# Autodesk Inventor assembly: ヘッケン＋揺動節2_MIR
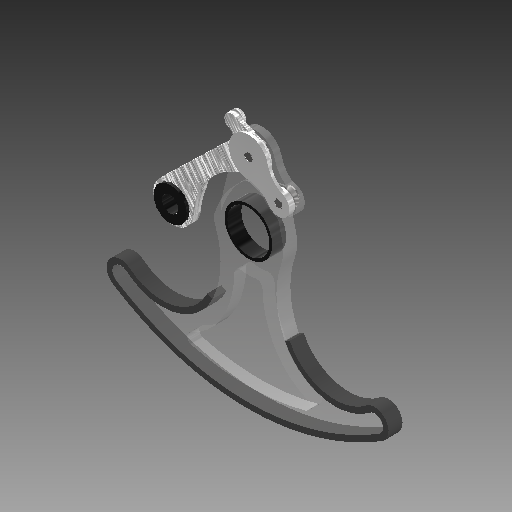
[picture p0: Inventor's stored thumbnail of the model, 512x512]
Saved by Autodesk Inventor 2020 (Build 240168000, 168)
## iProperties
Created: 2019-09-03
Part Number: ヘッケン＋揺動節2_MIR
Document SubType Name: Assembly
Designer: 雪村
Mass: 16.6288 g
Surface Area: 132.4 cm^2
Volume: 11.4961 cm^3
Density: 1.44647 g/cm^3
Author: 雪村
## Documents named in this file (9)
- C:\Users\white\Documents\SRDC\SRDC\Inventor_2017\2018年機体\2020年4年機体\ヘッケン＋揺動節2_MIR.iam
- C:\Users\white\Documents\SRDC\SRDC\Inventor_2017\2018年機体\パーツ\オイレス151705.ipt
- C:\Users\white\Documents\SRDC\SRDC\Inventor_2017\2018年機体\2020年4年機体\ヘッケン2_MIR.ipt
- C:\Users\white\Documents\SRDC\SRDC\Inventor_2017\2018年機体\2020年4年機体\脚揺動節1_MIR1.ipt
- C:\Users\white\Documents\SRDC\SRDC\Inventor_2017\2018年機体\2020年4年機体\脚ゴム2.ipt
- C:\Users\white\Documents\SRDC\SRDC\Inventor_2017\2018年機体\2020年4年機体\脚揺動節抑え1.ipt
- C:\Users\white\Documents\SRDC\SRDC\Inventor_2017\2018年機体\パーツ\オイレス060801.5.ipt
- C:\Users\white\Documents\SRDC\SRDC\Inventor_2017\2018年機体\パーツ\ネジ皿m3,05.ipt
- C:\Users\white\Documents\SRDC\SRDC\Inventor_2017\2018年機体\パーツ\オイレスフランジ付き06080512,1t.ipt
## Components (9 placed, 8 different names)
1. オイレス151705:1 — 挿入:4
2. ヘッケン2_MIR:1 — 挿入:1, 挿入:2, 挿入:4, 挿入:5, 挿入:6, 挿入:7, 挿入:8, 挿入:9
3. 脚揺動節1_MIR1:1 — 挿入:3, 挿入:10
4. 脚ゴム2:1 — 挿入:1, 挿入:2
5. 脚揺動節抑え1:1 — 挿入:6, 挿入:7
6. オイレス060801.5:1 — 挿入:3, 挿入:5
7. ネジ皿m3,05:1 — 挿入:8
8. ネジ皿m3,05:2 — 挿入:9
9. オイレスフランジ付き06080512,1t:1 — 挿入:10
## Relationships (10: Insert 10)
- 挿入:1 [Insert]: ヘッケン2_MIR:1 ↔ 脚ゴム2:1
- 挿入:2 [Insert]: ヘッケン2_MIR:1 ↔ 脚ゴム2:1
- 挿入:3 [Insert]: 脚揺動節1_MIR1:1 ↔ オイレス060801.5:1
- 挿入:4 [Insert]: オイレス151705:1 ↔ ヘッケン2_MIR:1
- 挿入:5 [Insert] (0.1 mm): ヘッケン2_MIR:1 ↔ オイレス060801.5:1
- 挿入:6 [Insert]: ヘッケン2_MIR:1 ↔ 脚揺動節抑え1:1
- 挿入:7 [Insert]: ヘッケン2_MIR:1 ↔ 脚揺動節抑え1:1
- 挿入:8 [Insert]: ヘッケン2_MIR:1 ↔ ネジ皿m3,05:1
- 挿入:9 [Insert]: ヘッケン2_MIR:1 ↔ ネジ皿m3,05:2
- 挿入:10 [Insert]: 脚揺動節1_MIR1:1 ↔ オイレスフランジ付き06080512,1t:1
